# Autodesk Inventor assembly: EnsamblePierna
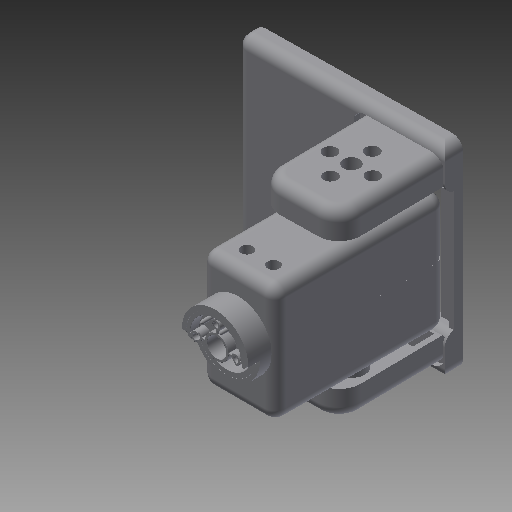
[picture p0: Inventor's stored thumbnail of the model, 512x512]
Saved by Autodesk Inventor 2019 (Build 230136000, 136)
## iProperties
Created: 2016-12-19
Part Number: EnsamblePierna
Document SubType Name: Assembly
Designer: Mario
Author: Mario
## Documents named in this file (6)
- D:\Documents\Kevin\robot\EnsamblePierna.iam
- D:\Documents\Kevin\robot\PiernaP1.ipt
- D:\Documents\Kevin\robot\SERVO.iam
- D:\Documents\Kevin\robot\PiernaP2.ipt
- D:\Documents\Kevin\robot\EnsamblePie.iam
- D:\Documents\Kevin\robot\EjeTobillo.ipt
## Components (5 placed, 5 different names)
1. PiernaP1:1
2. SERVO:1 [sub-assembly] — Insert:1
3. PiernaP2:1 — Insert:2
4. EnsamblePie:1 [sub-assembly] — Insert:1
5. EjeTobillo:1 — Insert:2
## Relationships (2: Insert 2)
- Insert:1: SERVO:1 ↔ EnsamblePie:1
- Insert:2: PiernaP2:1 ↔ EjeTobillo:1
